# Autodesk Inventor assembly: Prototype_02
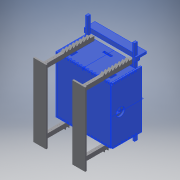
[picture p0: Inventor's stored thumbnail of the model, 180x180]
Saved by Autodesk Inventor 2019.4 (Build 234330000, 330)
## iProperties
Created: 2019-12-18
Part Number: Prototype_02
Document SubType Name: Assembly
Designer: fabfarm
Author: fabfarm
## Documents named in this file (3)
- D:\Users\fabfarm\Documents\Saw table\Prototype_02.iam
- D:\Users\fabfarm\Documents\Saw table\BOX_PART.iam
- D:\Users\fabfarm\Documents\Saw table\Static_foot_V02.iam
## Components (3 placed, 2 different names)
1. BOX_PART:1 [sub-assembly] — Flush:1, Mate:1, Flush:2, Mate:2, Flush:4
2. Static_foot_V02:1 [sub-assembly] — Flush:1, Mate:1, Flush:3, Flush:4
3. Static_foot_V02:2 [sub-assembly] — Flush:2, Flush:3, Mate:2
## Relationships (6: Flush 4, Mate 2)
- Flush:1: BOX_PART:1 ↔ Static_foot_V02:1
- Mate:1: BOX_PART:1 ↔ Static_foot_V02:1
- Flush:2: BOX_PART:1 ↔ Static_foot_V02:2
- Flush:3: Static_foot_V02:1 ↔ Static_foot_V02:2
- Mate:2: BOX_PART:1 ↔ Static_foot_V02:2
- Flush:4 (18.55 mm): BOX_PART:1 ↔ Static_foot_V02:1
